# Autodesk Inventor assembly: 後輪軸+後輪
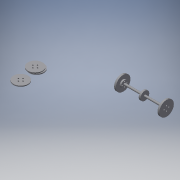
[picture p0: Inventor's stored thumbnail of the model, 180x180]
Saved by Autodesk Inventor 2019 (Build 230136000, 136)
## iProperties
Created: 2020-03-19
Part Number: 後輪軸+後輪
Material: 一般
Document SubType Name: Assembly
Designer: 黃柏維
Author: 黃柏維
## Documents named in this file (3)
- C:\Users\user\Desktop\機工實務\後輪軸+後輪.iam
- C:\Users\user\Desktop\機工實務\後輪.ipt
- C:\Users\user\Desktop\機工實務\煞車桿.ipt
## Components (8 placed, 2 different names)
1. 後輪:1 — 貼合:1, 插入:1, 貼合:4, 插入:4
2. 煞車桿:1 — 貼合:1, 插入:1, 貼合:2, 插入:2
3. 後輪:2 — 貼合:2, 插入:2, 貼合:3, 插入:3
4. 後輪:3
5. 後輪:4 — 貼合:3, 插入:3
6. 後輪:5 — 貼合:4, 插入:4
7. 後輪:6
8. 後輪:7
## Relationships (8: Mate 4, Insert 4)
- 貼合:1 [Mate]: 後輪:1 ↔ 煞車桿:1
- 插入:1 [Insert]: 後輪:1 ↔ 煞車桿:1
- 貼合:2 [Mate]: 煞車桿:1 ↔ 後輪:2
- 插入:2 [Insert]: 煞車桿:1 ↔ 後輪:2
- 貼合:3 [Mate]: 後輪:2 ↔ 後輪:4
- 插入:3 [Insert]: 後輪:2 ↔ 後輪:4
- 貼合:4 [Mate]: 後輪:1 ↔ 後輪:5
- 插入:4 [Insert]: 後輪:1 ↔ 後輪:5
